# Autodesk Inventor assembly: 13042026
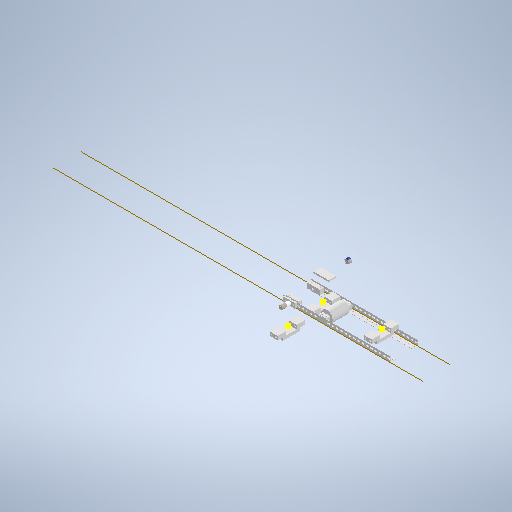
[picture p0: Inventor's stored thumbnail of the model, 512x512]
Saved by Autodesk Inventor 2025.2 (Build 292293000, 293)
## iProperties
Created: 2026-04-13
Part Number: 13042026
Document SubType Name: Assembly
Designer: Oski
Author: Oski
## Documents named in this file (15)
- C:\Users\Oski\Desktop\ProjektPrzejsciowy\Inventor\13042026\13042026.iam
- C:\Users\Oski\Desktop\ProjektPrzejsciowy\Inventor\13042026\Parts\28BYJ48 — kopia\28BYJ48 — kopia\28BYJ48 — kopia.ipt
- C:\Users\Oski\Desktop\ProjektPrzejsciowy\Inventor\13042026\Parts\13042025-02.ipt
- C:\Users\Oski\Desktop\ProjektPrzejsciowy\Inventor\13042026\Parts\706-2_6200ZZ_10x30x9mm_Groove_Ball_Bearing_STEP242\706-2_6200ZZ_10x30x9mm_Groove_Ball_Bearing_STEP242\706-2_6200ZZ_10x30x9mm_Groove_Ball_Bearing_.iam
- C:\Users\Oski\Desktop\ProjektPrzejsciowy\Inventor\13042026\Parts\706-2_6200ZZ_10x30x9mm_Groove_Ball_Bearing_STEP242\25d-metal-gearmotor-172-227\25d-metal-gearmotor-172-227\25d-metal-gearmotor-172-227.ipt
- C:\Users\Oski\Desktop\ProjektPrzejsciowy\Inventor\13042026\Parts\13042026-01.ipt
- C:\Users\Oski\Desktop\ProjektPrzejsciowy\Inventor\13042026\Parts\13042026-04.ipt
- C:\Users\Oski\Desktop\ProjektPrzejsciowy\Inventor\13042026\Parts\13042026-03.ipt
- C:\Users\Oski\Desktop\ProjektPrzejsciowy\Inventor\13042026\Parts\13042026-05.ipt
- C:\Users\Oski\Desktop\ProjektPrzejsciowy\Inventor\13042026\Parts\13042026-06.ipt
- C:\Users\Oski\Desktop\ProjektPrzejsciowy\Inventor\13042026\Parts\m8x40_din933.ipt
- C:\Users\Oski\Desktop\ProjektPrzejsciowy\Inventor\13042026\Parts\1883316.iam
- C:\Users\Oski\Desktop\ProjektPrzejsciowy\Inventor\13042026\Parts\13042026-07.ipt
- C:\Users\Oski\Desktop\ProjektPrzejsciowy\Inventor\13042026\Parts\13042026-09.ipt
- C:\Users\Oski\Desktop\ProjektPrzejsciowy\Inventor\13042026\Parts\13042026-08.ipt
## Components (21 placed, 14 different names)
1. 28BYJ48 — kopia:1
2. 13042025-02:1
3. 706-2_6200ZZ_10x30x9mm_Groove_Ball_Bearing_:1 [sub-assembly] — Insert:1, Rotational:2
4. 25d-metal-gearmotor-172-227:1 — Mate:19, Mate:20, Mate:21, Mate:22, Mate:23
5. 13042026-01:1 — Insert:1, Insert:3
6. 13042026-04:1 — Mate:24, Mate:25, Mate:26, Mate:27, Mate:28, Mate:29, Mate:30, Mate:31, Mate:32
7. 13042026-04:2 — Mate:2, Mate:3, Mate:4, Mate:5, Mate:6, Mate:7, Mate:8, Mate:9, Mate:10, Mate:11, Mate:13
8. 13042026-03:1 — Rotational:1, Mate:6, Mate:9, Mate:10, Mate:12, Mate:14
9. 706-2_6200ZZ_10x30x9mm_Groove_Ball_Bearing_:2 [sub-assembly] — Insert:3, Rotational:1
10. 13042026-03:2 — Rotational:2
11. 13042026-05:1 — Mate:2, Mate:3, Mate:4, Mate:5, Mate:25, Mate:26, Mate:27
12. 13042026-05:2
13. 13042026-05:3
14. 13042026-06:1 — Mate:7, Mate:8
15. m8x40_din933:1 — Mate:11, Mate:12
16. m8x40_din933:2 — Mate:13, Mate:14
17. 1883316:1 [sub-assembly] — Mate:17, Mate:18
18. 1883316:2 [sub-assembly] — Mate:15, Mate:16
19. 13042026-07:1 — Mate:15, Mate:16, Mate:17, Mate:18, Mate:24, Mate:28, Mate:29
20. 13042026-09:1 — Mate:19, Mate:20, Mate:21, Mate:30, Mate:31, Mate:32
21. 13042026-08:1 — Mate:22, Mate:23
## Relationships (35: Mate 31, Insert 2, RevoluteJoint 2)
- Insert:1: 706-2_6200ZZ_10x30x9mm_Groove_Ball_Bearing_:1 ↔ 13042026-01:1
- Insert:3: 13042026-01:1 ↔ 706-2_6200ZZ_10x30x9mm_Groove_Ball_Bearing_:2
- Rotational:1 [RevoluteJoint]: 13042026-03:1 ↔ 706-2_6200ZZ_10x30x9mm_Groove_Ball_Bearing_:2
- Rotational:2 [RevoluteJoint]: 706-2_6200ZZ_10x30x9mm_Groove_Ball_Bearing_:1 ↔ 13042026-03:2
- Mate:2: 13042026-04:2 ↔ 13042026-05:1
- Mate:3: 13042026-04:2 ↔ 13042026-05:1
- Mate:4: 13042026-04:2 ↔ 13042026-05:1
- Mate:5: 13042026-04:2 ↔ 13042026-05:1
- Mate:6: 13042026-04:2 ↔ 13042026-03:1
- Mate:7: 13042026-04:2 ↔ 13042026-06:1
- Mate:8: 13042026-04:2 ↔ 13042026-06:1
- Mate:9: 13042026-04:2 ↔ 13042026-03:1
- Mate:10: 13042026-04:2 ↔ 13042026-03:1
- Mate:11: 13042026-04:2 ↔ m8x40_din933:1
- Mate:12: 13042026-03:1 ↔ m8x40_din933:1
- Mate:13: 13042026-04:2 ↔ m8x40_din933:2
- Mate:14: 13042026-03:1 ↔ m8x40_din933:2
- Mate:15: 1883316:2 ↔ 13042026-07:1
- Mate:16: 1883316:2 ↔ 13042026-07:1
- Mate:17: 1883316:1 ↔ 13042026-07:1
- Mate:18: 1883316:1 ↔ 13042026-07:1
- Mate:19: 25d-metal-gearmotor-172-227:1 ↔ 13042026-09:1
- Mate:20: 25d-metal-gearmotor-172-227:1 ↔ 13042026-09:1
- Mate:21: 25d-metal-gearmotor-172-227:1 ↔ 13042026-09:1
- Mate:22: 25d-metal-gearmotor-172-227:1 ↔ 13042026-08:1
- Mate:23: 25d-metal-gearmotor-172-227:1 ↔ 13042026-08:1
- Mate:24: 13042026-04:1 ↔ 13042026-07:1
- Mate:25: 13042026-04:1 ↔ 13042026-05:1
- Mate:26: 13042026-04:1 ↔ 13042026-05:1
- Mate:27: 13042026-04:1 ↔ 13042026-05:1
- Mate:28: 13042026-04:1 ↔ 13042026-07:1
- Mate:29: 13042026-04:1 ↔ 13042026-07:1
- Mate:30: 13042026-04:1 ↔ 13042026-09:1
- Mate:31: 13042026-04:1 ↔ 13042026-09:1
- Mate:32: 13042026-04:1 ↔ 13042026-09:1
